# Autodesk Inventor assembly: sl2
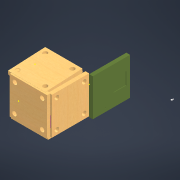
[picture p0: Inventor's stored thumbnail of the model, 180x180]
Saved by Autodesk Inventor 2021 (Build 250183000, 183)
## iProperties
Created: 2021-06-25
Part Number: sl2
Document SubType Name: Assembly
Designer: Acer
Author: Acer
## Documents named in this file (10)
- C:\Users\Mohammed Khalid\Documents\locker (1).iam
- C:\Users\Mohammed Khalid\Documents\side (4).ipt
- C:\Users\Mohammed Khalid\Documents\B.ipt
- C:\Users\Mohammed Khalid\Documents\l clamp.ipt
- C:\Users\Mohammed Khalid\Documents\front view.ipt
- C:\Users\Mohammed Khalid\Documents\plank.ipt
- C:\Users\Mohammed Khalid\Documents\TOWER BOLT CASING (1).ipt
- C:\Users\Mohammed Khalid\Documents\BOLT (1).ipt
- C:\Users\Mohammed Khalid\Documents\TOWER BOLT LOCK (2).ipt
- C:\Users\Mohammed Khalid\Documents\Pan Head Screw.ipt
## Components (16 placed, 9 different names)
1. side (4):1 — Mate:1, Mate:3, Mate:5
2. side (4):2 — Mate:2, Mate:4
3. side (4):3 — Mate:1, Mate:2, Flush:1, Mate:6, Angle:1
4. B:2 — Mate:3
5. side (4):4 — Flush:1, Mate:7
6. l clamp:1
7. side (4):5 — Mate:4
8. front view:1 — Mate:5, Angle:1
9. plank:1 — Mate:6
10. TOWER BOLT LOCK (2):1
11. Pan Head Screw:1
12. Pan Head Screw:2
13. Pan Head Screw:3
14. Pan Head Screw:4
15. TOWER BOLT CASING (1):2 — Mate:7, Insert:1
16. BOLT (1):3 — Insert:1
## Relationships (10: Mate 7, Flush 1, Angle 1, Insert 1)
- Mate:1: side (4):1 ↔ side (4):3
- Mate:2: side (4):2 ↔ side (4):3
- Flush:1: side (4):3 ↔ side (4):4
- Mate:3: side (4):1 ↔ B:2
- Mate:4: side (4):2 ↔ side (4):5
- Mate:5: side (4):1 ↔ front view:1
- Mate:6: side (4):3 ↔ plank:1
- Angle:1 (-90 deg): side (4):3 ↔ front view:1
- Mate:7: side (4):4 ↔ TOWER BOLT CASING (1):2
- Insert:1: TOWER BOLT CASING (1):2 ↔ BOLT (1):3
